# Autodesk Inventor assembly: mg996r_rot_frame
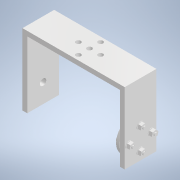
[picture p0: Inventor's stored thumbnail of the model, 180x180]
Saved by Autodesk Inventor 2021.4 (Build 254397000, 397)
## iProperties
Created: 2022-08-02
Part Number: mg996r_rot_frame
Document SubType Name: Assembly
Designer: isamu
Author: isamu
## Documents named in this file (6)
- D:\personal_projects\robot\inventor\2021_matlab_compat _v2\servo_rot_frame\mg996r_rot_frame.iam
- D:\personal_projects\robot\inventor\2021_matlab_compat _v2\servo_frames\servo_handle.iam
- D:\personal_projects\robot\exports\frames\servo frame mg996r.ipt
- D:\personal_projects\robot\exports\screws\m2 nuts.ipt
- D:\personal_projects\robot\exports\screws\m2 washer.ipt
- D:\personal_projects\robot\exports\screws\m4 nuts.ipt
## Components (11 placed, 5 different names)
1. servo_handle:1 [sub-assembly] — Mate:1, Mate:2, Mate:3
2. servo frame mg996r:1 — Mate:1, Mate:2, Mate:3, Insert:5, Insert:6, Insert:7, Insert:8, Insert:13
3. m2 nuts:1 — Insert:10
4. m2 nuts:2 — Insert:12
5. m2 nuts:3 — Insert:11
6. m2 nuts:4 — Insert:9
7. m2 washer:1 — Insert:6, Insert:9
8. m2 washer:2 — Insert:5, Insert:10
9. m2 washer:3 — Insert:8, Insert:11
10. m2 washer:4 — Insert:7, Insert:12
11. m4 nuts:1 — Insert:13
## Relationships (12: Insert 9, Mate 3)
- Mate:1: servo_handle:1 ↔ servo frame mg996r:1
- Mate:2: servo_handle:1 ↔ servo frame mg996r:1
- Mate:3: servo_handle:1 ↔ servo frame mg996r:1
- Insert:5: servo frame mg996r:1 ↔ m2 washer:2
- Insert:6: servo frame mg996r:1 ↔ m2 washer:1
- Insert:7: servo frame mg996r:1 ↔ m2 washer:4
- Insert:8: servo frame mg996r:1 ↔ m2 washer:3
- Insert:9: m2 nuts:4 ↔ m2 washer:1
- Insert:10: m2 nuts:1 ↔ m2 washer:2
- Insert:11: m2 nuts:3 ↔ m2 washer:3
- Insert:12: m2 nuts:2 ↔ m2 washer:4
- Insert:13: servo frame mg996r:1 ↔ m4 nuts:1
